# Autodesk Inventor assembly: ring_assembly
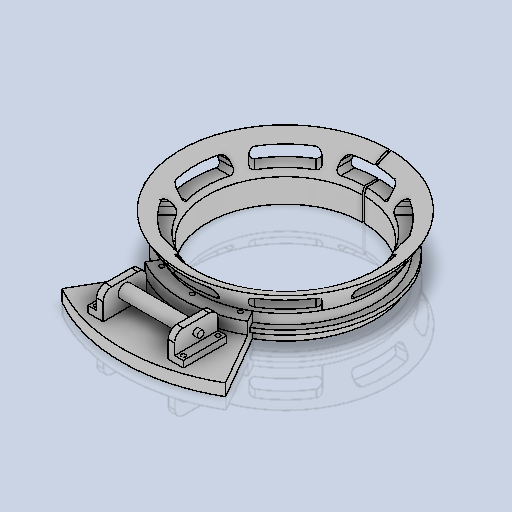
[picture p0: Inventor's stored thumbnail of the model, 512x512]
Saved by Autodesk Inventor 2026.1 (Build 301233000, 233)
## iProperties
Created: 2025-08-31
Part Number: ring_assembly
Document SubType Name: Assembly
Designer: baseb
Author: baseb
## Documents named in this file (5)
- C:\Users\baseb\Desktop\LANL-Glovebox-Closure-Mechanism\ring_assembly.iam
- C:\Users\baseb\Desktop\LANL-Glovebox-Closure-Mechanism\Glove_ring.ipt
- C:\Users\baseb\Desktop\LANL-Glovebox-Closure-Mechanism\shelf_attachment.ipt
- C:\Users\baseb\Desktop\LANL-Glovebox-Closure-Mechanism\drum_holder.ipt
- C:\Users\baseb\Desktop\LANL-Glovebox-Closure-Mechanism\drum.ipt
## Components (5 placed, 4 different names)
1. Glove_ring:1 — Mate:1, Flush:1
2. shelf_attachment:1 — Mate:1, Flush:1, Mate:2, Mate:3, Mate:4, Mate:5, Mate:6, Mate:7
3. drum_holder:1 — Mate:5, Mate:6, Mate:7
4. drum_holder:2 — Mate:2, Mate:3, Mate:4, Mate:8, Mate:9
5. drum:1 — Mate:8, Mate:9
## Relationships (10: Mate 9, Flush 1)
- Mate:1: Glove_ring:1 ↔ shelf_attachment:1
- Flush:1: Glove_ring:1 ↔ shelf_attachment:1
- Mate:2: shelf_attachment:1 ↔ drum_holder:2
- Mate:3: shelf_attachment:1 ↔ drum_holder:2
- Mate:4: shelf_attachment:1 ↔ drum_holder:2
- Mate:5: shelf_attachment:1 ↔ drum_holder:1
- Mate:6: shelf_attachment:1 ↔ drum_holder:1
- Mate:7: shelf_attachment:1 ↔ drum_holder:1
- Mate:8: drum_holder:2 ↔ drum:1
- Mate:9: drum_holder:2 ↔ drum:1
